# Autodesk Inventor assembly: 000-dribl-v2
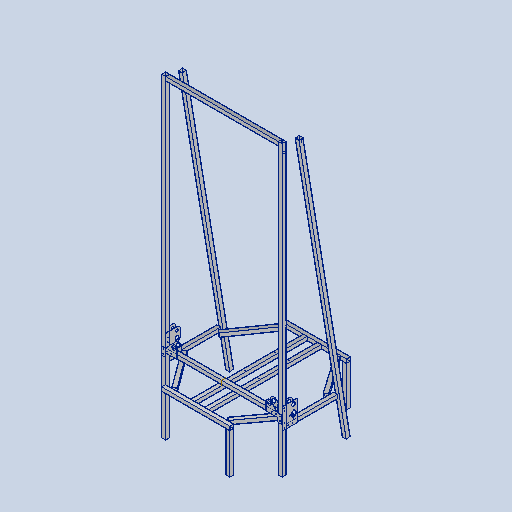
[picture p0: Inventor's stored thumbnail of the model, 512x512]
Saved by Autodesk Inventor 2025.2 (Build 292293000, 293)
## iProperties
Created: 2025-04-03
Part Number: 000-dribl-v2
Document SubType Name: Assembly
Designer: haruy
Author: haruy
## Documents named in this file (6)
- C:\Users\haruy\Documents\ロボコン\NHK2025\cad\nagahisa\dribl\000-dribl-v2.iam
- C:\Users\haruy\Documents\ロボコン\NHK2025\cad\nagahisa\dribl\dribl-v3-Sketch-Base.ipt
- C:\Users\haruy\Documents\ロボコン\NHK2025\cad\nagahisa\dribl\dribl-v1-Plate-2.ipt
- C:\Users\haruy\Documents\ロボコン\NHK2025\cad\nagahisa\dribl\dribl-v1-Plate-5.ipt
- C:\Users\haruy\Documents\ロボコン\NHK2025\cad\nagahisa\dribl\dribl-v1-Plate-3.ipt
- C:\Users\haruy\Documents\ロボコン\NHK2025\cad\nagahisa\dribl\dribl-v1-Plate-4.ipt
## Components (9 placed, 5 different names)
1. dribl-v3-Sketch-Base:1 — 挿入:1, 挿入:2, 挿入:3, 挿入:4, 挿入:5, 挿入:6, 挿入:7, 挿入:8, 挿入:9, 挿入:10, 挿入:11, 挿入:12, 挿入:13, 挿入:14, 挿入:15, 挿入:16, 挿入:17
2. dribl-v1-Plate-2:1 — 挿入:1, 挿入:2, 挿入:3
3. dribl-v1-Plate-2:2 — 挿入:4, 挿入:5
4. dribl-v1-Plate-2:3 — 挿入:8, 挿入:9
5. dribl-v1-Plate-2:4 — 挿入:6, 挿入:7
6. dribl-v1-Plate-5:1 — 挿入:12, 挿入:13
7. dribl-v1-Plate-5:2 — 挿入:10, 挿入:11
8. dribl-v1-Plate-3:1 — 挿入:14, 挿入:15
9. dribl-v1-Plate-4:1 — 挿入:16, 挿入:17
## Relationships (17: Insert 17)
- 挿入:1 [Insert]: dribl-v3-Sketch-Base:1 ↔ dribl-v1-Plate-2:1
- 挿入:2 [Insert]: dribl-v3-Sketch-Base:1 ↔ dribl-v1-Plate-2:1
- 挿入:3 [Insert]: dribl-v3-Sketch-Base:1 ↔ dribl-v1-Plate-2:1
- 挿入:4 [Insert]: dribl-v3-Sketch-Base:1 ↔ dribl-v1-Plate-2:2
- 挿入:5 [Insert]: dribl-v3-Sketch-Base:1 ↔ dribl-v1-Plate-2:2
- 挿入:6 [Insert]: dribl-v3-Sketch-Base:1 ↔ dribl-v1-Plate-2:4
- 挿入:7 [Insert]: dribl-v3-Sketch-Base:1 ↔ dribl-v1-Plate-2:4
- 挿入:8 [Insert]: dribl-v3-Sketch-Base:1 ↔ dribl-v1-Plate-2:3
- 挿入:9 [Insert]: dribl-v3-Sketch-Base:1 ↔ dribl-v1-Plate-2:3
- 挿入:10 [Insert]: dribl-v3-Sketch-Base:1 ↔ dribl-v1-Plate-5:2
- 挿入:11 [Insert]: dribl-v3-Sketch-Base:1 ↔ dribl-v1-Plate-5:2
- 挿入:12 [Insert]: dribl-v3-Sketch-Base:1 ↔ dribl-v1-Plate-5:1
- 挿入:13 [Insert]: dribl-v3-Sketch-Base:1 ↔ dribl-v1-Plate-5:1
- 挿入:14 [Insert]: dribl-v3-Sketch-Base:1 ↔ dribl-v1-Plate-3:1
- 挿入:15 [Insert]: dribl-v3-Sketch-Base:1 ↔ dribl-v1-Plate-3:1
- 挿入:16 [Insert]: dribl-v3-Sketch-Base:1 ↔ dribl-v1-Plate-4:1
- 挿入:17 [Insert]: dribl-v3-Sketch-Base:1 ↔ dribl-v1-Plate-4:1
